# Autodesk Inventor assembly: Head
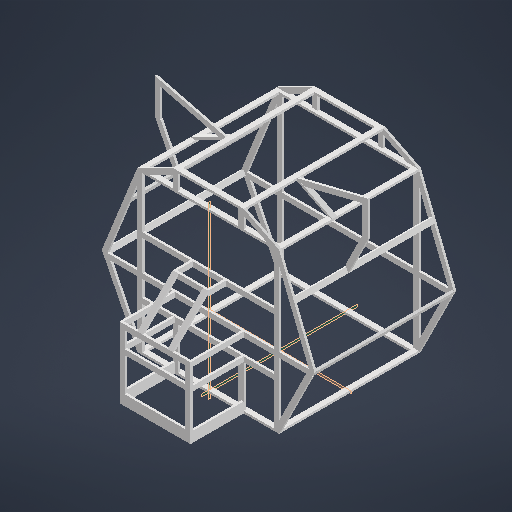
[picture p0: Inventor's stored thumbnail of the model, 512x512]
Saved by Autodesk Inventor 2026 (Build 300175000, 175)
## iProperties
Created: 2025-09-02
Part Number: Head
Document SubType Name: Assembly
Designer: trott
Author: trott
## Documents named in this file (23)
- C:\Users\trott\Documents\UofSC-ASME-Tiger-Burn-Design-2025\CAD\Head\Head.iam
- C:\Users\trott\Documents\UofSC-ASME-Tiger-Burn-Design-2025\CAD\Head\2x4x96.ipt
- C:\Users\trott\Documents\UofSC-ASME-Tiger-Burn-Design-2025\CAD\Head\2x4x89.ipt
- C:\Users\trott\Documents\UofSC-ASME-Tiger-Burn-Design-2025\CAD\Head\2x4x105.ipt
- C:\Users\trott\Documents\UofSC-ASME-Tiger-Burn-Design-2025\CAD\Head\S_2x4x24.ipt
- C:\Users\trott\Documents\UofSC-ASME-Tiger-Burn-Design-2025\CAD\Head\S_2x4x64.622.ipt
- C:\Users\trott\Documents\UofSC-ASME-Tiger-Burn-Design-2025\CAD\Head\S_2x4x48.13.ipt
- C:\Users\trott\Documents\UofSC-ASME-Tiger-Burn-Design-2025\CAD\Head\2x4x48.ipt
- C:\Users\trott\Documents\UofSC-ASME-Tiger-Burn-Design-2025\CAD\Head\2x4x10.5.ipt
- C:\Users\trott\Documents\UofSC-ASME-Tiger-Burn-Design-2025\CAD\Head\S_2x4x26.833.ipt
- C:\Users\trott\Documents\UofSC-ASME-Tiger-Burn-Design-2025\CAD\Head\2x4x93.ipt
- C:\Users\trott\Documents\UofSC-ASME-Tiger-Burn-Design-2025\CAD\Head\S2_2x4x26.833.ipt
- C:\Users\trott\Documents\UofSC-ASME-Tiger-Burn-Design-2025\CAD\Head\S_2x4x45.87.ipt
- C:\Users\trott\Documents\UofSC-ASME-Tiger-Burn-Design-2025\CAD\Head\S2_2x4x24.ipt
- C:\Users\trott\Documents\UofSC-ASME-Tiger-Burn-Design-2025\CAD\Head\S_2x4x29.814.ipt
- C:\Users\trott\Documents\UofSC-ASME-Tiger-Burn-Design-2025\CAD\Head\2x4x12.ipt
- C:\Users\trott\Documents\UofSC-ASME-Tiger-Burn-Design-2025\CAD\Head\2x4x36.ipt
- C:\Users\trott\Documents\UofSC-ASME-Tiger-Burn-Design-2025\CAD\Head\2x4x45.ipt
- C:\Users\trott\Documents\UofSC-ASME-Tiger-Burn-Design-2025\CAD\Head\2x4x28.5.ipt
- C:\Users\trott\Documents\UofSC-ASME-Tiger-Burn-Design-2025\CAD\Head\2x4x11.ipt
- C:\Users\trott\Documents\UofSC-ASME-Tiger-Burn-Design-2025\CAD\Head\2x4x21.ipt
- C:\Users\trott\Documents\UofSC-ASME-Tiger-Burn-Design-2025\CAD\Head\2x4x23.ipt
- C:\Users\trott\Documents\UofSC-ASME-Tiger-Burn-Design-2025\CAD\Head\S_2x4x33.941.ipt
## Components (75 placed, 22 different names)
1. 2x4x89:5 — Mate:5, Flush:11, Flush:12, Flush:14, Flush:15, Flush:18, Flush:23, Flush:24, Flush:52, Mate:62, Flush:75, Mate:64, Flush:79, Mate:71
2. 2x4x89:6 — Mate:6, Flush:13, Flush:14
3. S_2x4x64.622:1 — Mate:9, Flush:19
4. S_2x4x64.622:2 — Mate:10, Flush:20, Mate:46, Flush:58
5. S_2x4x64.622:3 — Mate:11, Mate:12, Flush:21, Mate:41, Mate:45, Flush:57
6. S_2x4x64.622:4 — Mate:13, Mate:14
7. S_2x4x48.13:1 — Mate:15, Flush:22, Mate:16
8. S_2x4x48.13:2 — Mate:17, Flush:25
9. S_2x4x48.13:3 — Mate:18, Mate:19, Flush:26, Mate:40
10. S_2x4x48.13:4 — Mate:20, Mate:21, Flush:27
11. 2x4x10.5:1 — Mate:22, Flush:28, Flush:32, Flush:39, Flush:40, Mate:27, Flush:46
12. 2x4x10.5:2 — Mate:23, Flush:29, Flush:31, Flush:45
13. 2x4x10.5:3 — Mate:24, Flush:34, Flush:35, Flush:38, Flush:47
14. 2x4x10.5:4 — Mate:25, Flush:33, Flush:36, Flush:37, Mate:26, Flush:48
15. 2x4x48:1 — Flush:37, Flush:38, Mate:26, Flush:41, Mate:28, Flush:42, Mate:33, Mate:35
16. 2x4x48:2 — Flush:39, Flush:40, Mate:27, Flush:43, Flush:44, Mate:29, Mate:30, Mate:31
17. 2x4x89:7 — Flush:41, Mate:28, Flush:42, Mate:43, Mate:55
18. 2x4x89:8 — Flush:43, Flush:44, Mate:29, Mate:42, Mate:53
19. S_2x4x26.833:1 — Flush:45, Mate:30, Flush:56
20. S_2x4x26.833:2 — Mate:31, Mate:32, Flush:46, Flush:55
21. S_2x4x26.833:3 — Mate:33, Mate:34, Flush:47
22. S_2x4x26.833:4 — Mate:35, Flush:48
23. 2x4x89:10 — Mate:37, Flush:51, Flush:52, Mate:84, Flush:116, Flush:118, Mate:85, Flush:120
24. 2x4x93:1 — Mate:38, Mate:39, Flush:53
25. 2x4x93:2 — Mate:40, Mate:41, Flush:54
26. S2_2x4x26.833:1 — Mate:42, Flush:56, Flush:67, Flush:68, Flush:70
27. S2_2x4x26.833:2 — Mate:43, Mate:44, Flush:55, Mate:56, Flush:71
28. 2x4x93:3 — Mate:45, Flush:57, Mate:61
29. 2x4x93:4 — Mate:46, Flush:58
30. S2_2x4x24:1 — Flush:65, Flush:66, Flush:67, Flush:69, Mate:54
31. S_2x4x45.87:1 — Mate:53, Flush:68, Flush:69
32. S_2x4x29.814:1 — Mate:54, Flush:70
33. S_2x4x45.87:2 — Mate:55, Mate:56, Flush:71, Mate:57, Mate:58, Flush:72, Flush:73
34. S2_2x4x24:2 — Mate:57, Mate:58, Flush:72, Flush:73, Mate:59, Mate:60, Flush:74
35. S_2x4x29.814:2 — Mate:59, Mate:60, Flush:74, Mate:61
36. 2x4x36:1 — Mate:62, Flush:75, Mate:68, Flush:83, Flush:84, Flush:92, Flush:114, Flush:115
37. 2x4x36:2 — Mate:64, Flush:79, Flush:90, Flush:113
38. 2x4x45:1 — Mate:68, Flush:83, Flush:84, Mate:82
39. 2x4x36:3 — Mate:72, Flush:89, Flush:90, Flush:94, Flush:98, Mate:87, Flush:128
40. 2x4x89:11 — Mate:70, Flush:87, Mate:71, Mate:72, Flush:89, Mate:73, Flush:91
41. 2x4x36:4 — Mate:73, Flush:91, Flush:92, Flush:96, Mate:76, Flush:97, Flush:125, Flush:126
42. 2x4x36:5 — Mate:74, Flush:93, Flush:94, Flush:100, Mate:78, Flush:101, Flush:102, Flush:109
43. 2x4x36:6 — Mate:75, Flush:95, Flush:96, Mate:77, Flush:99, Flush:103, Flush:104, Flush:111
44. 2x4x45:3 — Mate:76, Flush:97, Flush:98, Flush:112, Mate:83, Flush:124
45. 2x4x45:4 — Mate:77, Flush:99, Flush:100, Flush:107
46. 2x4x36:7 — Mate:78, Flush:101, Flush:102, Flush:105, Flush:106, Mate:79
47. 2x4x36:8 — Flush:103, Flush:104, Flush:105
48. 2x4x45:5 — Flush:106, Mate:79, Flush:107
49. 2x4x28.5:1 — Flush:108, Mate:80, Flush:109
50. 2x4x28.5:2 — Flush:110, Mate:81, Flush:111
51. 2x4x11:1 — Mate:82, Flush:112, Flush:113, Flush:127
52. 2x4x11:2 — Mate:83, Flush:114, Flush:115
53. 2x4x12:1 — Mate:84, Flush:116, Flush:118, Flush:119, Mate:86, Flush:122, Flush:123, Flush:131
54. 2x4x12:2 — Mate:85, Flush:120, Flush:121
55. 2x4x21:1 — Mate:86, Flush:122, Flush:123, Mate:91, Mate:92
56. 2x4x23:1 — Flush:124, Flush:125, Flush:126
57. 2x4x23:2 — Flush:127, Mate:87, Flush:128
58. S_2x4x33.941:1 — Mate:91, Flush:131
59. S_2x4x33.941:2 — Mate:92
60. 2x4x105:1 — Mate:4, Flush:9, Flush:10, Mate:5, Flush:11, Mate:8, Flush:17, Mate:19, Flush:26, Flush:87, Flush:117
61. 2x4x105:2 — Mate:6, Flush:13, Mate:20, Flush:27
62. 2x4x105:3 — Mate:7, Flush:16, Flush:22, Mate:37, Flush:51, Mate:70
63. 2x4x105:4 — Flush:25
64. 2x4x96:1 — Mate:1, Flush:1, Flush:2, Mate:2, Flush:3, Flush:4, Mate:4, Flush:9, Flush:10, Mate:21, Flush:88
65. 2x4x89:1 — Mate:1, Flush:1, Flush:2, Flush:8
66. 2x4x89:2 — Mate:2, Flush:3, Flush:4, Flush:5, Mate:3, Flush:6, Flush:7, Flush:12, Flush:77, Mate:74, Flush:93, Mate:75, Flush:95, Flush:108, Mate:80, Flush:110, Mate:81
67. 2x4x96:2 — Flush:5, Mate:3, Flush:6, Flush:7, Flush:8, Mate:15, Mate:16
68. 2x4x96:3 — Mate:12, Mate:13, Flush:32, Flush:35, Mate:32, Mate:34, Mate:44
69. 2x4x89:3 — Mate:24, Mate:25, Flush:33, Flush:34
70. 2x4x89:4 — Mate:22, Mate:23, Flush:28, Flush:29
71. 2x4x96:4 — Flush:31, Flush:36, Flush:65, Flush:66
72. S_2x4x24:2 — Mate:8, Flush:17, Flush:18, Mate:11, Flush:21, Flush:24, Mate:18, Flush:54
73. S_2x4x24:1 — Mate:7, Flush:15, Flush:16, Mate:10, Flush:20, Flush:23, Mate:38, Mate:39, Flush:53
74. S_2x4x24:3 — Mate:14
75. S_2x4x24:4 — Mate:9, Flush:19, Mate:17
## Component patterns: (4 elements, first: 2x4x105:1), (2 elements, first: 2x4x96:1 + 2x4x89:1 + 2x4x89:2 + 2x4x96:2), (2 elements, first: S_2x4x24:2 + S_2x4x24:1)
## Relationships (190: Flush 113, Mate 77)
- Mate:1: 2x4x96:1 ↔ 2x4x89:1
- Flush:1: 2x4x96:1 ↔ 2x4x89:1
- Flush:2: 2x4x96:1 ↔ 2x4x89:1
- Mate:2: 2x4x96:1 ↔ 2x4x89:2
- Flush:3: 2x4x96:1 ↔ 2x4x89:2
- Flush:4: 2x4x96:1 ↔ 2x4x89:2
- Flush:5: 2x4x89:2 ↔ 2x4x96:2
- Mate:3: 2x4x89:2 ↔ 2x4x96:2
- Flush:6: 2x4x89:2 ↔ 2x4x96:2
- Flush:7: 2x4x89:2 ↔ 2x4x96:2
- Flush:8: 2x4x89:1 ↔ 2x4x96:2
- Mate:4: 2x4x105:1 ↔ 2x4x96:1
- Flush:9: 2x4x105:1 ↔ 2x4x96:1
- Flush:10: 2x4x105:1 ↔ 2x4x96:1
- Mate:5: 2x4x89:5 ↔ 2x4x105:1
- Flush:11: 2x4x89:5 ↔ 2x4x105:1
- Flush:12 (1130.3 mm): 2x4x89:5 ↔ 2x4x89:2
- Mate:6: 2x4x89:6 ↔ 2x4x105:2
- Flush:13: 2x4x89:6 ↔ 2x4x105:2
- Flush:14: 2x4x89:5 ↔ 2x4x89:6
- Mate:7: 2x4x105:3 ↔ S_2x4x24:1
- Flush:15: 2x4x89:5 ↔ S_2x4x24:1
- Flush:16: 2x4x105:3 ↔ S_2x4x24:1
- Mate:8: 2x4x105:1 ↔ S_2x4x24:2
- Flush:17: 2x4x105:1 ↔ S_2x4x24:2
- Flush:18: 2x4x89:5 ↔ S_2x4x24:2
- Mate:9: S_2x4x64.622:1 ↔ S_2x4x24:4
- Flush:19: S_2x4x64.622:1 ↔ S_2x4x24:4
- Mate:10: S_2x4x64.622:2 ↔ S_2x4x24:1
- Flush:20: S_2x4x64.622:2 ↔ S_2x4x24:1
- Mate:11: S_2x4x64.622:3 ↔ S_2x4x24:2
- Mate:12: S_2x4x64.622:3 ↔ 2x4x96:3
- Flush:21: S_2x4x64.622:3 ↔ S_2x4x24:2
- Mate:13: S_2x4x64.622:4 ↔ 2x4x96:3
- Mate:14: S_2x4x64.622:4 ↔ S_2x4x24:3
- Mate:15: S_2x4x48.13:1 ↔ 2x4x96:2
- Flush:22: S_2x4x48.13:1 ↔ 2x4x105:3
- Mate:16: S_2x4x48.13:1 ↔ 2x4x96:2
- Flush:23: 2x4x89:5 ↔ S_2x4x24:1
- Flush:24: 2x4x89:5 ↔ S_2x4x24:2
- Mate:17: S_2x4x48.13:2 ↔ S_2x4x24:4
- Flush:25: S_2x4x48.13:2 ↔ 2x4x105:4
- Mate:18: S_2x4x48.13:3 ↔ S_2x4x24:2
- Mate:19: S_2x4x48.13:3 ↔ 2x4x105:1
- Flush:26: S_2x4x48.13:3 ↔ 2x4x105:1
- Mate:20: S_2x4x48.13:4 ↔ 2x4x105:2
- Mate:21: S_2x4x48.13:4 ↔ 2x4x96:1
- Flush:27: S_2x4x48.13:4 ↔ 2x4x105:2
- Mate:22: 2x4x10.5:1 ↔ 2x4x89:4
- Mate:23: 2x4x10.5:2 ↔ 2x4x89:4
- Flush:28: 2x4x10.5:1 ↔ 2x4x89:4
- Flush:29: 2x4x10.5:2 ↔ 2x4x89:4
- Flush:31 (609.6 mm): 2x4x10.5:2 ↔ 2x4x96:4
- Flush:32 (609.6 mm): 2x4x10.5:1 ↔ 2x4x96:3
- Mate:24: 2x4x10.5:3 ↔ 2x4x89:3
- Mate:25: 2x4x10.5:4 ↔ 2x4x89:3
- Flush:33: 2x4x10.5:4 ↔ 2x4x89:3
- Flush:34: 2x4x10.5:3 ↔ 2x4x89:3
- Flush:35 (609.6 mm): 2x4x10.5:3 ↔ 2x4x96:3
- Flush:36 (609.6 mm): 2x4x10.5:4 ↔ 2x4x96:4
- Flush:37: 2x4x10.5:4 ↔ 2x4x48:1
- Flush:38: 2x4x10.5:3 ↔ 2x4x48:1
- Mate:26: 2x4x10.5:4 ↔ 2x4x48:1
- Flush:39: 2x4x10.5:1 ↔ 2x4x48:2
- Flush:40: 2x4x10.5:1 ↔ 2x4x48:2
- Mate:27: 2x4x10.5:1 ↔ 2x4x48:2
- Flush:41: 2x4x48:1 ↔ 2x4x89:7
- Mate:28: 2x4x48:1 ↔ 2x4x89:7
- Flush:42: 2x4x48:1 ↔ 2x4x89:7
- Flush:43: 2x4x48:2 ↔ 2x4x89:8
- Flush:44: 2x4x48:2 ↔ 2x4x89:8
- Mate:29: 2x4x48:2 ↔ 2x4x89:8
- Flush:45: 2x4x10.5:2 ↔ S_2x4x26.833:1
- Mate:30: 2x4x48:2 ↔ S_2x4x26.833:1
- Mate:31: 2x4x48:2 ↔ S_2x4x26.833:2
- Mate:32: S_2x4x26.833:2 ↔ 2x4x96:3
- Flush:46: 2x4x10.5:1 ↔ S_2x4x26.833:2
- Mate:33: 2x4x48:1 ↔ S_2x4x26.833:3
- Mate:34: S_2x4x26.833:3 ↔ 2x4x96:3
- Flush:47: 2x4x10.5:3 ↔ S_2x4x26.833:3
- Mate:35: 2x4x48:1 ↔ S_2x4x26.833:4
- Flush:48: 2x4x10.5:4 ↔ S_2x4x26.833:4
- Mate:37: 2x4x89:10 ↔ 2x4x105:3
- Flush:51: 2x4x89:10 ↔ 2x4x105:3
- Flush:52 (-609.6 mm): 2x4x89:5 ↔ 2x4x89:10
- Mate:38: 2x4x93:1 ↔ S_2x4x24:1
- Mate:39: 2x4x93:1 ↔ S_2x4x24:1
- Flush:53: 2x4x93:1 ↔ S_2x4x24:1
- Mate:40: S_2x4x48.13:3 ↔ 2x4x93:2
- Mate:41: S_2x4x64.622:3 ↔ 2x4x93:2
- Flush:54: 2x4x93:2 ↔ S_2x4x24:2
- Mate:42: 2x4x89:8 ↔ S2_2x4x26.833:1
- Mate:43: 2x4x89:7 ↔ S2_2x4x26.833:2
- Mate:44: S2_2x4x26.833:2 ↔ 2x4x96:3
- Flush:55 (914.4 mm): S_2x4x26.833:2 ↔ S2_2x4x26.833:2
- Flush:56 (914.4 mm): S_2x4x26.833:1 ↔ S2_2x4x26.833:1
- Mate:45: S_2x4x64.622:3 ↔ 2x4x93:3
- Flush:57: S_2x4x64.622:3 ↔ 2x4x93:3
- Mate:46: S_2x4x64.622:2 ↔ 2x4x93:4
- Flush:58: S_2x4x64.622:2 ↔ 2x4x93:4
- Flush:65 (-609.6 mm): S2_2x4x24:1 ↔ 2x4x96:4
- Flush:66 (38.1 mm): S2_2x4x24:1 ↔ 2x4x96:4
- Flush:67: S2_2x4x26.833:1 ↔ S2_2x4x24:1
- Mate:53: 2x4x89:8 ↔ S_2x4x45.87:1
- Flush:68: S2_2x4x26.833:1 ↔ S_2x4x45.87:1
- Flush:69: S2_2x4x24:1 ↔ S_2x4x45.87:1
- Mate:54: S2_2x4x24:1 ↔ S_2x4x29.814:1
- Flush:70: S2_2x4x26.833:1 ↔ S_2x4x29.814:1
- Mate:55: 2x4x89:7 ↔ S_2x4x45.87:2
- Mate:56: S2_2x4x26.833:2 ↔ S_2x4x45.87:2
- Flush:71: S2_2x4x26.833:2 ↔ S_2x4x45.87:2
- Mate:57: S_2x4x45.87:2 ↔ S2_2x4x24:2
- Mate:58: S_2x4x45.87:2 ↔ S2_2x4x24:2
- Flush:72: S_2x4x45.87:2 ↔ S2_2x4x24:2
- Flush:73: S_2x4x45.87:2 ↔ S2_2x4x24:2
- Mate:59: S2_2x4x24:2 ↔ S_2x4x29.814:2
- Mate:60: S2_2x4x24:2 ↔ S_2x4x29.814:2
- Flush:74: S2_2x4x24:2 ↔ S_2x4x29.814:2
- Mate:61: 2x4x93:3 ↔ S_2x4x29.814:2
- Mate:62: 2x4x89:5 ↔ 2x4x36:1
- Flush:75: 2x4x89:5 ↔ 2x4x36:1
- Flush:77 (-1219.2 mm): 2x4x89:2
- Mate:64: 2x4x89:5 ↔ 2x4x36:2
- Flush:79: 2x4x89:5 ↔ 2x4x36:2
- Mate:68: 2x4x36:1 ↔ 2x4x45:1
- Flush:83: 2x4x36:1 ↔ 2x4x45:1
- Flush:84: 2x4x36:1 ↔ 2x4x45:1
- Mate:70: 2x4x89:11 ↔ 2x4x105:3
- Flush:87: 2x4x89:11 ↔ 2x4x105:1
- Mate:71 (-457.2 mm): 2x4x89:5 ↔ 2x4x89:11
- Flush:88 (-1219.2 mm): 2x4x96:1
- Mate:72: 2x4x36:3 ↔ 2x4x89:11
- Flush:89: 2x4x36:3 ↔ 2x4x89:11
- Flush:90: 2x4x36:2 ↔ 2x4x36:3
- Mate:73: 2x4x89:11 ↔ 2x4x36:4
- Flush:91: 2x4x89:11 ↔ 2x4x36:4
- Flush:92: 2x4x36:1 ↔ 2x4x36:4
- Mate:74: 2x4x36:5 ↔ 2x4x89:2
- Flush:93: 2x4x36:5 ↔ 2x4x89:2
- Flush:94: 2x4x36:3 ↔ 2x4x36:5
- Mate:75: 2x4x36:6 ↔ 2x4x89:2
- Flush:95: 2x4x36:6 ↔ 2x4x89:2
- Flush:96: 2x4x36:4 ↔ 2x4x36:6
- Mate:76: 2x4x36:4 ↔ 2x4x45:3
- Flush:97: 2x4x36:4 ↔ 2x4x45:3
- Flush:98: 2x4x36:3 ↔ 2x4x45:3
- Mate:77: 2x4x36:6 ↔ 2x4x45:4
- Flush:99: 2x4x36:6 ↔ 2x4x45:4
- Flush:100: 2x4x36:5 ↔ 2x4x45:4
- Mate:78 (-177.8 mm): 2x4x36:5 ↔ 2x4x36:7
- Flush:101: 2x4x36:5 ↔ 2x4x36:7
- Flush:102: 2x4x36:5 ↔ 2x4x36:7
- Flush:103: 2x4x36:6 ↔ 2x4x36:8
- Flush:104: 2x4x36:6 ↔ 2x4x36:8
- Flush:105: 2x4x36:7 ↔ 2x4x36:8
- Flush:106: 2x4x36:7 ↔ 2x4x45:5
- Mate:79: 2x4x36:7 ↔ 2x4x45:5
- Flush:107: 2x4x45:4 ↔ 2x4x45:5
- Flush:108: 2x4x28.5:1 ↔ 2x4x89:2
- Mate:80: 2x4x28.5:1 ↔ 2x4x89:2
- Flush:109: 2x4x36:5 ↔ 2x4x28.5:1
- Flush:110: 2x4x28.5:2 ↔ 2x4x89:2
- Mate:81: 2x4x28.5:2 ↔ 2x4x89:2
- Flush:111: 2x4x36:6 ↔ 2x4x28.5:2
- Mate:82: 2x4x45:1 ↔ 2x4x11:1
- Flush:112: 2x4x45:3 ↔ 2x4x11:1
- Flush:113: 2x4x36:2 ↔ 2x4x11:1
- Mate:83: 2x4x45:3 ↔ 2x4x11:2
- Flush:114: 2x4x36:1 ↔ 2x4x11:2
- Flush:115: 2x4x36:1 ↔ 2x4x11:2
- Mate:84: 2x4x89:10 ↔ 2x4x12:1
- Flush:116: 2x4x89:10 ↔ 2x4x12:1
- Flush:117 (-1219.2 mm): 2x4x105:1
- Flush:118: 2x4x89:10 ↔ 2x4x12:1
- Flush:119 (-304.8 mm): 2x4x12:1
- Mate:85: 2x4x89:10 ↔ 2x4x12:2
- Flush:120: 2x4x89:10 ↔ 2x4x12:2
- Flush:121 (-304.8 mm): 2x4x12:2
- Mate:86: 2x4x12:1 ↔ 2x4x21:1
- Flush:122: 2x4x12:1 ↔ 2x4x21:1
- Flush:123: 2x4x12:1 ↔ 2x4x21:1
- Flush:124: 2x4x45:3 ↔ 2x4x23:1
- Flush:125: 2x4x36:4 ↔ 2x4x23:1
- Flush:126: 2x4x36:4 ↔ 2x4x23:1
- Flush:127: 2x4x11:1 ↔ 2x4x23:2
- Mate:87: 2x4x36:3 ↔ 2x4x23:2
- Flush:128: 2x4x36:3 ↔ 2x4x23:2
- Mate:91: 2x4x21:1 ↔ S_2x4x33.941:1
- Flush:131: 2x4x12:1 ↔ S_2x4x33.941:1
- Mate:92: 2x4x21:1 ↔ S_2x4x33.941:2
